# Autodesk Inventor assembly: Pressure Vessel, Global Assembly
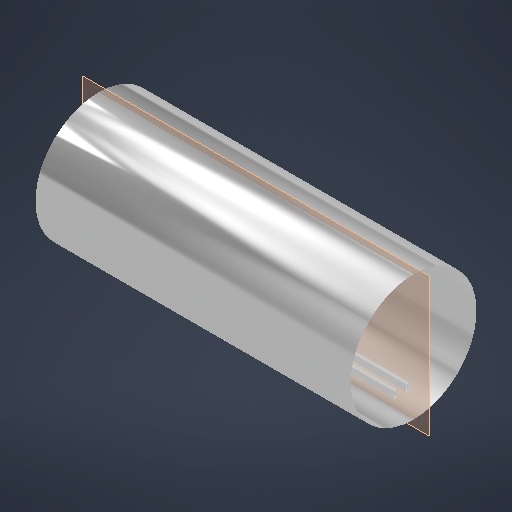
[picture p0: Inventor's stored thumbnail of the model, 512x512]
Saved by Autodesk Inventor 2026 (Build 300175000, 175)
## iProperties
Created: 2025-10-25
Part Number: Pressure Vessel, Global Assembly
Document SubType Name: Assembly
Designer: Brandon Portillo
Author: Brandon Portillo
## Documents named in this file (3)
- C:\Users\anarc\GitHub\TSGC-NASA_Senior_Design\CAD\Pressure Vessel\Pressure Vessel, Global Assembly.iam
- C:\Users\anarc\GitHub\TSGC-NASA_Senior_Design\CAD\Pressure Vessel\Pressure Vessel, Single Part.ipt
- C:\Users\anarc\GitHub\TSGC-NASA_Senior_Design\CAD\Pressure Vessel\Box Beam.ipt
## Components (3 placed, 2 different names)
1. Pressure Vessel, Single Part:1 — Flush:1, Flush:2
2. Box Beam:1 — Flush:2, Flush:3
3. Box Beam:2 — Flush:1, Flush:3
## Relationships (3: Flush 3)
- Flush:1: Pressure Vessel, Single Part:1 ↔ Box Beam:2
- Flush:2: Pressure Vessel, Single Part:1 ↔ Box Beam:1
- Flush:3: Box Beam:1 ↔ Box Beam:2
